# Autodesk Inventor assembly: Wheel Orientation
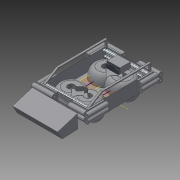
[picture p0: Inventor's stored thumbnail of the model, 180x180]
Saved by Autodesk Inventor 2015 (Build 190159000, 159)
## iProperties
Created: 2016-01-19
Part Number: Wheel Orientation
Document SubType Name: Assembly
Designer: sethbattis
Author: sethbattis
## Documents named in this file (12)
- \\area51\team3566\cad\FRC 2016\Space Claims.iam
- \\area51\team3566\cad\FRC 2016\Wheelbase.ipt
- \\area51\team3566\cad\FRC 2016\Basic Frame.ipt
- \\area51\team3566\cad\FRC 2016\Corner Bumper.ipt
- \\area51\team3566\cad\FRC 2016\AM14U3 End Sheet 24.5in.ipt
- \\area51\team3566\cad\FRC 2016\Roll Bar.ipt
- \\area51\team3566\cad\FRC 2016\Floor.ipt
- \\area51\team3566\cad\FRC 2016\Imported Components\fc16-036_Battery.iam\fc16-036_Battery.iam.iam
- \\area51\team3566\cad\FRC 2016\Prow.ipt
- \\area51\team3566\cad\FRC 2016\Snow Blower Tire with Gear Box and Mini-CIM.iam
- \\area51\team3566\cad\FRC 2016\Snow Blower Tire with Gear Box and Mini-CIM_MIR.iam
- fc16-036_Battery.iam
## Components (17 placed, 10 different names)
1. Basic Frame:1 — Flush:1, Rigid:1, Mate:1, Mate:2, Flush:2, Flush:3, Flush:4, Flush:5, Mate:3, Mate:4, Flush:6, Flush:7, Flush:8, Flush:9, Mate:5, Flush:10, Mate:10, Mate:11, Mate:12, Flush:11, Flush:12, Flush:13, Flush:14, Flush:15, Rigid:2
2. Wheelbase:1 — Flush:1, Rigid:1, Rotational:1, Rotational:2, Rotational:3, Rotational:4
3. AM14U3 End Sheet 24.5in:1 — Flush:10, Mate:10
4. AM14U3 End Sheet 24.5in:2 — Mate:5, Mate:11
5. Floor:1 — Rigid:2, Mate:13
6. fc16-036_Battery.iam:1 [sub-assembly] — Mate:13
7. Prow:1
8. Corner Bumper:1 — Mate:1, Mate:3, Flush:6
9. Corner Bumper:2 — Mate:2, Flush:2, Flush:7
10. Corner Bumper:3 — Flush:4, Mate:4, Flush:9
11. Corner Bumper:4 — Flush:3, Flush:5, Flush:8
12. Roll Bar:1 — Flush:12, Flush:13, Flush:15
13. Roll Bar:2 — Mate:12, Flush:11, Flush:14
14. Snow Blower Tire with Gear Box and Mini-CIM:1 [sub-assembly] — Rotational:1
15. Snow Blower Tire with Gear Box and Mini-CIM:2 [sub-assembly] — Rotational:2
16. Snow Blower Tire with Gear Box and Mini-CIM_MIR:1 [sub-assembly] — Rotational:4
17. Snow Blower Tire with Gear Box and Mini-CIM_MIR:2 [sub-assembly] — Rotational:3
## Relationships (30: Flush 15, Mate 9, RevoluteJoint 4, WeldJoint 2)
- Flush:1: Basic Frame:1 ↔ Wheelbase:1
- Rigid:1 [WeldJoint]: Basic Frame:1 ↔ Wheelbase:1
- Mate:1: Basic Frame:1 ↔ Corner Bumper:1
- Mate:2: Basic Frame:1 ↔ Corner Bumper:2
- Flush:2: Basic Frame:1 ↔ Corner Bumper:2
- Flush:3: Basic Frame:1 ↔ Corner Bumper:4
- Flush:4: Basic Frame:1 ↔ Corner Bumper:3
- Flush:5: Basic Frame:1 ↔ Corner Bumper:4
- Mate:3: Basic Frame:1 ↔ Corner Bumper:1
- Mate:4: Basic Frame:1 ↔ Corner Bumper:3
- Flush:6: Basic Frame:1 ↔ Corner Bumper:1
- Flush:7: Basic Frame:1 ↔ Corner Bumper:2
- Flush:8: Basic Frame:1 ↔ Corner Bumper:4
- Flush:9: Basic Frame:1 ↔ Corner Bumper:3
- Mate:5: Basic Frame:1 ↔ AM14U3 End Sheet 24.5in:2
- Flush:10: Basic Frame:1 ↔ AM14U3 End Sheet 24.5in:1
- Mate:10: Basic Frame:1 ↔ AM14U3 End Sheet 24.5in:1
- Mate:11: Basic Frame:1 ↔ AM14U3 End Sheet 24.5in:2
- Mate:12: Basic Frame:1 ↔ Roll Bar:2
- Flush:11: Basic Frame:1 ↔ Roll Bar:2
- Flush:12: Basic Frame:1 ↔ Roll Bar:1
- Flush:13: Basic Frame:1 ↔ Roll Bar:1
- Flush:14: Basic Frame:1 ↔ Roll Bar:2
- Flush:15: Basic Frame:1 ↔ Roll Bar:1
- Rigid:2 [WeldJoint]: Basic Frame:1 ↔ Floor:1
- Mate:13: Floor:1 ↔ fc16-036_Battery.iam:1
- Rotational:1 [RevoluteJoint]: Wheelbase:1 ↔ Snow Blower Tire with Gear Box and Mini-CIM:1
- Rotational:2 [RevoluteJoint]: Wheelbase:1 ↔ Snow Blower Tire with Gear Box and Mini-CIM:2
- Rotational:3 [RevoluteJoint]: Wheelbase:1 ↔ Snow Blower Tire with Gear Box and Mini-CIM_MIR:2
- Rotational:4 [RevoluteJoint]: Wheelbase:1 ↔ Snow Blower Tire with Gear Box and Mini-CIM_MIR:1
